# Autodesk Inventor assembly: Pi4 Case Assembly
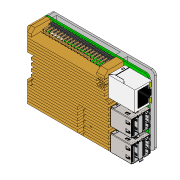
[picture p0: Inventor's stored thumbnail of the model, 180x180]
Saved by Autodesk Inventor 2020 (Build 240168000, 168)
## iProperties
Created: 2020-02-12
Part Number: Pi4 Case Assembly
Document SubType Name: Assembly
Designer: ahamm
Author: ahamm
## Documents named in this file (4)
- C:\Users\ahamm\Desktop\Inventor 2020 Parts\Inventor Download\Pi4 Case Assembly.iam
- C:\Users\ahamm\Desktop\Inventor 2020 Parts\Inventor Download\Raspberry Pi 4 Complete_Shrinkwrap_1.ipt
- C:\Users\ahamm\Desktop\Inventor 2020 Parts\Inventor Download\Heat sink.ipt
- C:\Users\ahamm\Desktop\Inventor 2020 Parts\Inventor Download\Heatsink Base.ipt
## Components (3 placed, 3 different names)
1. Raspberry Pi 4 Complete_Shrinkwrap_1:1 — Flush:1, Flush:2
2. Heat sink:1 — Flush:1, Flush:2, Flush:3
3. Heatsink Base:1 — Flush:3
## Relationships (3: Flush 3)
- Flush:1: Raspberry Pi 4 Complete_Shrinkwrap_1:1 ↔ Heat sink:1
- Flush:2: Raspberry Pi 4 Complete_Shrinkwrap_1:1 ↔ Heat sink:1
- Flush:3: Heat sink:1 ↔ Heatsink Base:1
